# Autodesk Inventor assembly: Y-Endstop-Holder
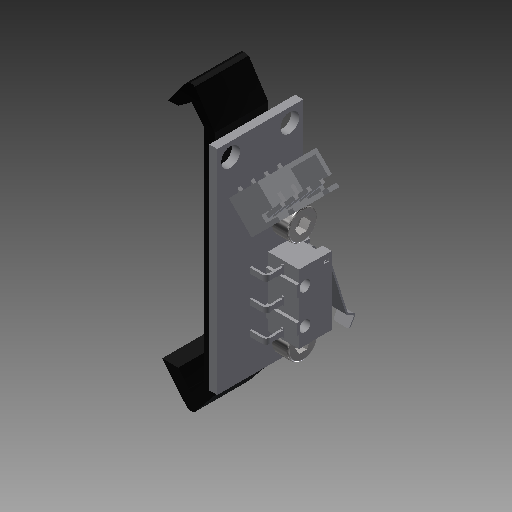
[picture p0: Inventor's stored thumbnail of the model, 512x512]
Saved by Autodesk Inventor 2018 (Build 220112000, 112)
## iProperties
Created: 2016-08-22
Part Number: Y-Endstop-Holder
Document SubType Name: Assembly
Designer: User
Author: User
## Documents named in this file (5)
- C:\Users\Dan\OneDrive\SL-Inventor\The Beast v1.2 PackandGo\Workspaces\Workspace\Y-Endstop-Holder.iam
- C:\Users\Dan\OneDrive\SL-Inventor\The Beast v1.2 PackandGo\Workspaces\Workspace\Y Endstop Holder.ipt
- C:\Users\Dan\OneDrive\SL-Inventor\The Beast v1.2 PackandGo\Workspaces\Workspace\en-US\CSN EN 24 036\CSN EN 24 036 - M3.ipt
- C:\Users\Dan\OneDrive\SL-Inventor\The Beast v1.2 PackandGo\Workspaces\Workspace\Capteur fin de course.ipt
- C:\Users\Dan\OneDrive\SL-Inventor\The Beast v1.2 PackandGo\Workspaces\Workspace\en-US\ANSI B18.3.1M(6)\ANSI B18.3.1M - M3x0.5 x 10(1).ipt
## Components (6 placed, 4 different names)
1. Y Endstop Holder:1
2. CSN EN 24036 M3:1
3. CSN EN 24036 M3:2
4. Capteur fin de course:1
5. Forged Socket Head Cap Screw - Metric M3x0.5 x 10:2
6. Forged Socket Head Cap Screw - Metric M3x0.5 x 10:1
## Relationships (10: Mate 7, Insert 2, Flush 1)
- [Mate]: Y Endstop Holder:1 ↔ CSN EN 24036 M3:1
- [Mate]: Y Endstop Holder:1 ↔ CSN EN 24036 M3:1
- [Mate]: Y Endstop Holder:1 ↔ CSN EN 24036 M3:1
- [Mate]: Y Endstop Holder:1 ↔ CSN EN 24036 M3:2
- [Mate]: Y Endstop Holder:1 ↔ CSN EN 24036 M3:2
- [Mate]: Y Endstop Holder:1 ↔ Capteur fin de course:1
- [Flush]: Y Endstop Holder:1 ↔ Capteur fin de course:1
- [Insert]: Capteur fin de course:1 ↔ Forged Socket Head Cap Screw - Metric M3x0.5 x 10:2
- [Insert]: Capteur fin de course:1 ↔ Forged Socket Head Cap Screw - Metric M3x0.5 x 10:1
- [Mate]: CSN EN 24036 M3:2 ↔ Forged Socket Head Cap Screw - Metric M3x0.5 x 10:1
